# Autodesk Inventor assembly: 1_Body
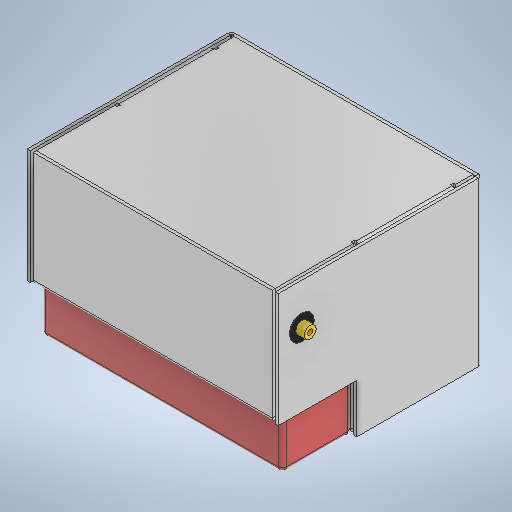
[picture p0: Inventor's stored thumbnail of the model, 512x512]
Saved by Autodesk Inventor 2025.2 (Build 292293000, 293)
## iProperties
Created: 2025-05-30
Part Number: 1_Body
Document SubType Name: Assembly
Designer: chris
Author: chris
## Documents named in this file (12)
- C:\Users\chris\문서\Inventor\RHp_Humanoid_ver1\Assembly\1_Body.iam
- C:\Users\chris\문서\Inventor\RHp_Humanoid_ver1\Part\Frame\Body\body_main_frame.ipt
- C:\Users\chris\문서\Inventor\RHp_Humanoid_ver1\Part\Frame\Body\body_back_frame.ipt
- C:\Users\chris\문서\Inventor\RHp_Humanoid_ver1\Part\Frame\Body\body_front_frame.ipt
- C:\Users\chris\문서\Inventor\RHp_Humanoid_ver1\Part\Frame\Body\body_middle_frame.ipt
- C:\Users\chris\문서\Inventor\RHp_Humanoid_ver1\Part\Frame\Body\body_motor_L_frame.ipt
- C:\Users\chris\문서\Inventor\RHp_Humanoid_ver1\Part\Frame\Body\body_motor_R_frame.ipt
- C:\Users\chris\문서\Inventor\RHp_Humanoid_ver1\Part\Frame\Body\body_top_frame.ipt
- C:\Users\chris\문서\Inventor\RHp_Humanoid_ver1\Part\HTD-45H, Horn\HTD-45H\HTD-45H.iam
- C:\Users\chris\문서\Inventor\RHp_Humanoid_ver1\Part\Frame\Body\Servo_Driver.ipt
- C:\Users\chris\문서\Inventor\RHp_Humanoid_ver1\Part\Frame\Body\Battery_Pack.ipt
- C:\Users\chris\문서\Inventor\P3766-P3768SKU4-P3767ENVELOPE\jetson_orin_super.iam
## Components (12 placed, 11 different names)
1. body_main_frame:1 — Mate:1, Mate:2, Flush:1, Mate:3, Flush:2, Mate:4, Mate:5, Flush:3, Flush:4, Mate:6, Flush:5, Mate:8, Mate:10, Mate:11, Flush:9, Flush:10, Mate:16, Mate:18, Flush:13, Mate:21, Mate:23
2. body_back_frame:1 — Mate:3, Flush:2, Mate:4, Mate:19
3. body_front_frame:1 — Mate:5, Flush:3, Flush:4, Flush:6, Mate:7, Flush:7, Mate:9, Flush:8
4. body_middle_frame:1 — Mate:6, Flush:5, Flush:6, Flush:11, Mate:13, Flush:12, Mate:15, Mate:17, Mate:22
5. body_motor_L_frame:1 — Mate:7, Flush:7, Mate:8, Mate:12
6. body_motor_R_frame:1 — Mate:9, Mate:10, Flush:8, Mate:14
7. body_top_frame:1 — Mate:11, Flush:9, Flush:10, Mate:20
8. HTD-45H:1 [sub-assembly] — Mate:12, Flush:11, Mate:13
9. HTD-45H:2 [sub-assembly] — Mate:14, Flush:12, Mate:15
10. Servo_Driver:1 — Mate:16, Mate:17, Mate:18
11. Battery_Pack:1 — Mate:19, Mate:20, Flush:13
12. jetson_orin_super:1 [sub-assembly] — Mate:21, Mate:22, Mate:23
## Relationships (36: Mate 23, Flush 13)
- Mate:1: body_main_frame:1
- Mate:2: body_main_frame:1
- Flush:1: body_main_frame:1
- Mate:3: body_main_frame:1 ↔ body_back_frame:1
- Flush:2: body_main_frame:1 ↔ body_back_frame:1
- Mate:4: body_main_frame:1 ↔ body_back_frame:1
- Mate:5: body_main_frame:1 ↔ body_front_frame:1
- Flush:3 (1.5 mm): body_main_frame:1 ↔ body_front_frame:1
- Flush:4: body_main_frame:1 ↔ body_front_frame:1
- Mate:6: body_main_frame:1 ↔ body_middle_frame:1
- Flush:5 (1.5 mm): body_main_frame:1 ↔ body_middle_frame:1
- Flush:6 (-30 mm): body_front_frame:1 ↔ body_middle_frame:1
- Mate:7: body_front_frame:1 ↔ body_motor_L_frame:1
- Flush:7: body_front_frame:1 ↔ body_motor_L_frame:1
- Mate:8 (40 mm): body_main_frame:1 ↔ body_motor_L_frame:1
- Mate:9: body_front_frame:1 ↔ body_motor_R_frame:1
- Mate:10 (40 mm): body_main_frame:1 ↔ body_motor_R_frame:1
- Mate:11: body_main_frame:1 ↔ body_top_frame:1
- Flush:8: body_front_frame:1 ↔ body_motor_R_frame:1
- Flush:9: body_main_frame:1 ↔ body_top_frame:1
- Flush:10: body_main_frame:1 ↔ body_top_frame:1
- Mate:12: body_motor_L_frame:1 ↔ HTD-45H:1
- Flush:11: body_middle_frame:1 ↔ HTD-45H:1
- Mate:13: body_middle_frame:1 ↔ HTD-45H:1
- Mate:14: body_motor_R_frame:1 ↔ HTD-45H:2
- Flush:12: body_middle_frame:1 ↔ HTD-45H:2
- Mate:15: body_middle_frame:1 ↔ HTD-45H:2
- Mate:16: body_main_frame:1 ↔ Servo_Driver:1
- Mate:17: body_middle_frame:1 ↔ Servo_Driver:1
- Mate:18 (31 mm): body_main_frame:1 ↔ Servo_Driver:1
- Mate:19: body_back_frame:1 ↔ Battery_Pack:1
- Mate:20: body_top_frame:1 ↔ Battery_Pack:1
- Flush:13 (-2.5 mm): body_main_frame:1 ↔ Battery_Pack:1
- Mate:21 (5 mm): body_main_frame:1 ↔ jetson_orin_super:1
- Mate:22: body_middle_frame:1 ↔ jetson_orin_super:1
- Mate:23 (8.5 mm): body_main_frame:1 ↔ jetson_orin_super:1
